# Autodesk Inventor assembly: Rotrkopf
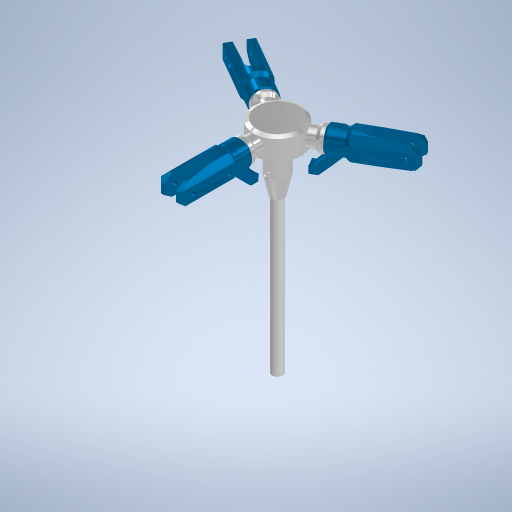
[picture p0: Inventor's stored thumbnail of the model, 512x512]
Saved by Autodesk Inventor 2023.2 (Build 272271000, 271)
## iProperties
Created: 2023-03-31
Part Number: Rotrkopf
Document SubType Name: Assembly
Designer: tadeu
Author: tadeu
## Documents named in this file (4)
- C:\Users\tadeu\Documents\0 Nerdy\CAD\Inventor\Studium\5. Semester\NWPL\WKA\Rotrkopf.iam
- C:\Users\tadeu\Documents\0 Nerdy\CAD\Inventor\Studium\5. Semester\NWPL\WKA\RotorKopf_Hub.ipt
- C:\Users\tadeu\Documents\0 Nerdy\CAD\Inventor\Studium\5. Semester\NWPL\WKA\RotorArm.ipt
- C:\Users\tadeu\Documents\0 Nerdy\CAD\Inventor\Studium\5. Semester\NWPL\WKA\Welle.ipt
## Components (5 placed, 3 different names)
1. RotorKopf_Hub:1 — Einfügen:1, Einfügen:2, Einfügen:3, Einfügen:4
2. RotorArm:1 — Einfügen:1
3. RotorArm:2 — Einfügen:2
4. RotorArm:3 — Einfügen:3
5. Welle:1 — Einfügen:4
## Relationships (4: Insert 4)
- Einfügen:1 [Insert]: RotorKopf_Hub:1 ↔ RotorArm:1
- Einfügen:2 [Insert]: RotorKopf_Hub:1 ↔ RotorArm:2
- Einfügen:3 [Insert]: RotorKopf_Hub:1 ↔ RotorArm:3
- Einfügen:4 [Insert]: RotorKopf_Hub:1 ↔ Welle:1
